# Autodesk Inventor assembly: CIM motor 12T thin
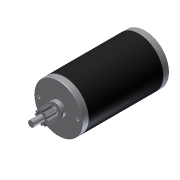
[picture p0: Inventor's stored thumbnail of the model, 180x180]
Saved by Autodesk Inventor 2011 (Build 150239000, 239)
## iProperties
Created: 2011-07-17
Part Number: CIM motor 12T thin
Document SubType Name: Assembly
Designer: Dan Niemitalo
Author: Dan Niemitalo
## Documents named in this file (4)
- H:\Nemo\Documents\Robotics\COTS Parts\Motors\CIM motor 12T.iam
- H:\Nemo\Documents\Robotics\Motors\CIM motor.ipt
- H:\Nemo\Documents\Robotics\Motors\2mmx2mmx10mm_key.ipt
- H:\Nemo\Documents\Robotics\COTS Parts\Gearboxes\Gears\Gear 20dp 8mm key 12T.ipt
## Components (3 placed, 3 different names)
1. CIM motor:1 — Mate:1, Angle:1, Mate:2, Mate:3, Mate:4
2. Spur Gear1:1 — Mate:1, Angle:1, Mate:2, Flush:1
3. 2mmx2mmx10mm_key:1 — Mate:3, Mate:4, Flush:1
## Relationships (6: Mate 4, Angle 1, Flush 1)
- Mate:1: CIM motor:1 ↔ Spur Gear1:1
- Angle:1 (0 deg): CIM motor:1 ↔ Spur Gear1:1
- Mate:2 (4.7625 mm): CIM motor:1 ↔ Spur Gear1:1
- Mate:3: CIM motor:1 ↔ 2mmx2mmx10mm_key:1
- Mate:4: CIM motor:1 ↔ 2mmx2mmx10mm_key:1
- Flush:1: Spur Gear1:1 ↔ 2mmx2mmx10mm_key:1
